# Autodesk Inventor assembly: Guidler Assembly
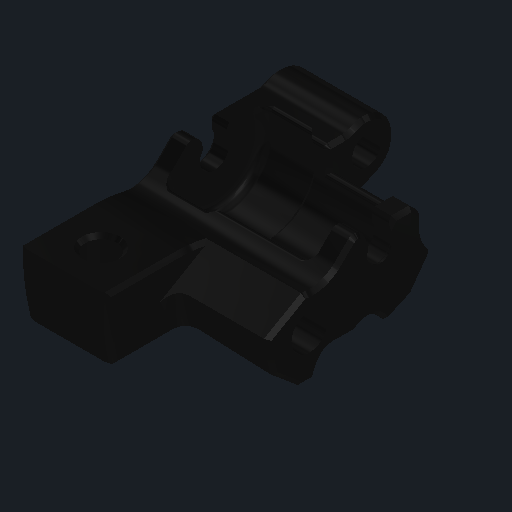
[picture p0: Inventor's stored thumbnail of the model, 512x512]
Saved by Autodesk Inventor 2025.1 (Build 291241020, 241B)
## iProperties
Created: 2025-05-11
Part Number: Guidler Assembly
Document SubType Name: Assembly
Designer: Joshua Eah
Author: Joshua Eah
## Documents named in this file (3)
- C:\Users\Joshua Eah\Documents\Voron 0.2\CAD\Master Assembly\Toolhead\Subassemblies\Guidler Assembly.iam
- C:\Users\Joshua Eah\Documents\Voron 0.2\CAD\Master Assembly\Hardware\M2x10 Self Tapper.ipt
- C:\Users\Joshua Eah\Documents\Voron 0.2\CAD\Master Assembly\Toolhead\Parts\Guidler.ipt
## Components (2 placed, 2 different names)
1. M2x10 Self Tapper:1
2. Guidler:1
## Relationships (1: Insert 1)
- [Insert]: M2x10 Self Tapper:1 ↔ Guidler:1
